# Autodesk Inventor assembly: Engine Assembly
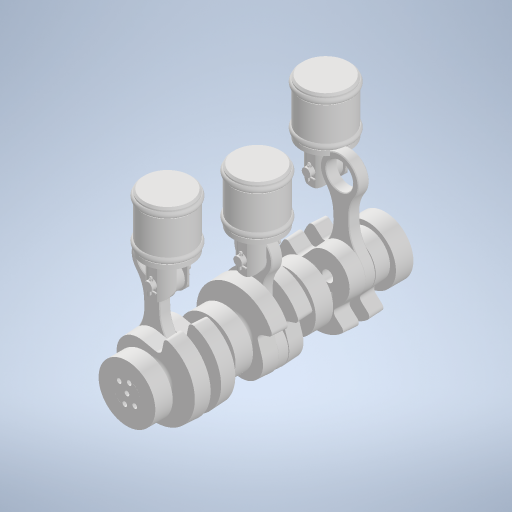
[picture p0: Inventor's stored thumbnail of the model, 512x512]
Saved by Autodesk Inventor 2023 (Build 270158000, 158)
## iProperties
Created: 2023-01-04
Part Number: Engine Assembly
Document SubType Name: Assembly
Designer: tgr41
Author: tgr41
## Documents named in this file (4)
- C:\Users\tgr41\OneDrive\Documents\Repositories\Steam-Engine\1.5x1 Inch 3 Cylidner\Cast Engine Block Design V4\Engine Assembly.iam
- C:\Users\tgr41\OneDrive\Documents\Repositories\Steam-Engine\1.5x1 Inch 3 Cylidner\Cast Engine Block Design V4\A.Crankshaft Subassembly.iam
- C:\Users\tgr41\OneDrive\Documents\Repositories\Steam-Engine\1.5x1 Inch 3 Cylidner\Cast Engine Block Design V4\A.Piston Subassembly.iam
- C:\Users\tgr41\OneDrive\Documents\Repositories\Steam-Engine\1.5x1 Inch 3 Cylidner\Cast Engine Block Design V4\C.Connecting Rod.ipt
## Components (7 placed, 3 different names)
1. A.Crankshaft Subassembly:1 [sub-assembly] — Mate:4, Mate:5, Mate:6, Mate:7, Mate:8, Mate:9
2. A.Piston Subassembly:1 [sub-assembly] — Mate:1
3. C.Connecting Rod:1 — Mate:1, Mate:4, Mate:9
4. A.Piston Subassembly:2 [sub-assembly]
5. C.Connecting Rod:2 — Mate:5, Mate:8
6. A.Piston Subassembly:3 [sub-assembly]
7. C.Connecting Rod:3 — Mate:6, Mate:7
## Relationships (9: Mate 9)
- Mate:1: A.Piston Subassembly:1 ↔ C.Connecting Rod:1
- [Mate]: A.Piston Subassembly:2 ↔ C.Connecting Rod:2
- [Mate]: A.Piston Subassembly:3 ↔ C.Connecting Rod:3
- Mate:4: A.Crankshaft Subassembly:1 ↔ C.Connecting Rod:1
- Mate:5: A.Crankshaft Subassembly:1 ↔ C.Connecting Rod:2
- Mate:6: A.Crankshaft Subassembly:1 ↔ C.Connecting Rod:3
- Mate:7: A.Crankshaft Subassembly:1 ↔ C.Connecting Rod:3
- Mate:8: A.Crankshaft Subassembly:1 ↔ C.Connecting Rod:2
- Mate:9: A.Crankshaft Subassembly:1 ↔ C.Connecting Rod:1
## Named parameters: d1_d0 = 0 mm, d2_d0 = 0 mm
